# Autodesk Inventor assembly: ArmDriver
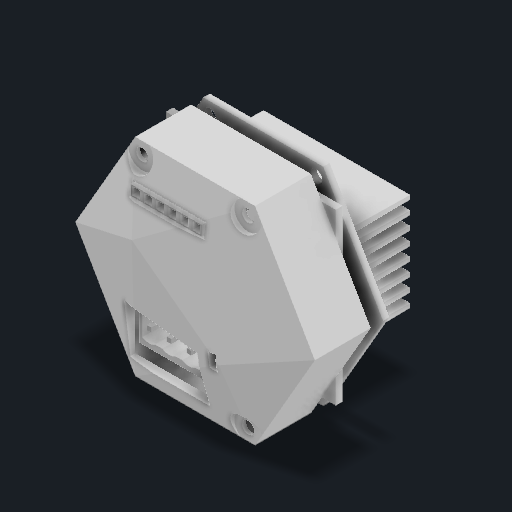
[picture p0: Inventor's stored thumbnail of the model, 512x512]
Saved by Autodesk Inventor 2025.2 (Build 292293000, 293)
## iProperties
Created: 2023-12-09
Part Number: ArmDriver
Document SubType Name: Assembly
Designer: valer
Author: valer
## Documents named in this file (4)
- C:\Users\valer\Desktop\str1ker\cad\ArmDriver.iam
- C:\Users\valer\Desktop\str1ker\cad\ArmDriverBoard.ipt
- C:\Users\valer\Desktop\str1ker\cad\external\ArmDriver\IBTMini.ipt
- C:\Users\valer\Desktop\str1ker\cad\ArmDriverBoardCover.ipt
## Components (3 placed, 3 different names)
1. ArmDriverBoard:1 — Mate:2, Mate:3, Mate:4
2. IBTMini:1 — Mate:2, Mate:3, Mate:4, Flush:1
3. ArmDriverBoardCover:1 — Flush:1
## Relationships (4: Mate 3, Flush 1)
- Mate:2: ArmDriverBoard:1 ↔ IBTMini:1
- Mate:3: ArmDriverBoard:1 ↔ IBTMini:1
- Mate:4: ArmDriverBoard:1 ↔ IBTMini:1
- Flush:1: IBTMini:1 ↔ ArmDriverBoardCover:1
